# Autodesk Inventor assembly: peg
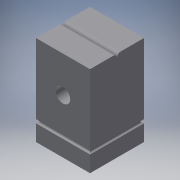
[picture p0: Inventor's stored thumbnail of the model, 180x180]
Saved by Autodesk Inventor 2019 (Build 230136000, 136)
## iProperties
Created: 2019-12-28
Part Number: peg
Material: Типовые
Document SubType Name: Assembly
Designer: stepa
Author: stepa
## Documents named in this file (2)
- C:\Users\stepa\Documents\Inventor\Shamisen\peg.iam
- C:\Users\stepa\Documents\Inventor\Shamisen\peg_half.ipt
## Components (2 placed, 1 different names)
1. peg_half:1 — Совмещение:1, Заподлицо:1, Заподлицо:2
2. peg_half:2 — Совмещение:1, Заподлицо:1, Заподлицо:2
## Relationships (3: Flush 2, Mate 1)
- Совмещение:1 [Mate]: peg_half:1 ↔ peg_half:2
- Заподлицо:1 [Flush]: peg_half:1 ↔ peg_half:2
- Заподлицо:2 [Flush]: peg_half:1 ↔ peg_half:2
